# Autodesk Inventor assembly: fabrication model end cap right
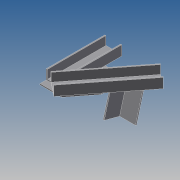
[picture p0: Inventor's stored thumbnail of the model, 180x180]
Saved by Autodesk Inventor 2014 SP1 (Build 180222100, 222)
## iProperties
Created: 2015-02-04
Part Number: fabrication model end cap right
Document SubType Name: Assembly
Designer: degan
Author: degan
## Documents named in this file (5)
- C:\Users\Dave\Desktop\hera-cad\support\endcaps\HERA_end_cap_right.iam
- C:\Users\Dave\Desktop\hera-cad\support\endcaps\angle channel.ipt
- C:\Users\Dave\Desktop\hera-cad\support\endcaps\side plate.ipt
- C:\Users\Dave\Desktop\hera-cad\support\endcaps\ring support right.ipt
- C:\Users\Dave\Desktop\hera-cad\support\endcaps\Horizontal channel right.ipt
## Components (4 placed, 4 different names)
1. ring support right:1 — Mate:4, Mate:5
2. angle channel:1 — Mate:1, Flush:1, Mate:3, Flush:2, Flush:3, Flush:5, Mate:4
3. Horizontal channel right:1 — Mate:1, Flush:1, Mate:2, Angle:1, Flush:4
4. side plate:1 — Flush:2, Flush:3, Flush:4, Flush:5, Mate:5
## Relationships (11: Mate 5, Flush 5, Angle 1)
- Mate:1: angle channel:1 ↔ Horizontal channel right:1
- Flush:1: angle channel:1 ↔ Horizontal channel right:1
- Mate:2: Horizontal channel right:1
- Angle:1 (90 deg): Horizontal channel right:1
- Mate:3: angle channel:1
- Flush:2: angle channel:1 ↔ side plate:1
- Flush:3: angle channel:1 ↔ side plate:1
- Flush:4: Horizontal channel right:1 ↔ side plate:1
- Flush:5: angle channel:1 ↔ side plate:1
- Mate:4: ring support right:1 ↔ angle channel:1
- Mate:5: ring support right:1 ↔ side plate:1
